# Autodesk Inventor assembly: Trunk
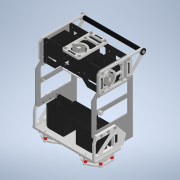
[picture p0: Inventor's stored thumbnail of the model, 180x180]
Saved by Autodesk Inventor 2020.4 (Build 244396000, 396)
## iProperties
Created: 2022-01-05
Part Number: Trunk
Document SubType Name: Assembly
Designer: Masato Kubotera
Author: Masato Kubotera
## Documents named in this file (25)
- C:\Users\Masato\Documents\Inventor\CIT Brains_Inventor\OpenPlatform_ver3_0 - ve4_1 branch\UpperBody\Trunk\Trunk.iam
- C:\Users\Masato\Documents\Inventor\CIT Brains_Inventor\OpenPlatform_ver3_0 - ve4_1 branch\Ready_Made\KONDO\B3M-SC-1040-A.ipt
- C:\Users\Masato\Documents\Inventor\CIT Brains_Inventor\OpenPlatform_ver3_0 - ve4_1 branch\Ready_Made\KONDO\B3M-SC-1170-A.ipt
- C:\Users\Masato\Documents\Inventor\CIT Brains_Inventor\OpenPlatform_ver3_0 - ve4_1 branch\UpperBody\Trunk\Trunk_chest_frame.ipt
- C:\Users\Masato\Documents\Inventor\CIT Brains_Inventor\OpenPlatform_ver3_0 - ve4_1 branch\Ready_Made\InsertNut\IRU-304SW.ipt
- C:\Users\Masato\Documents\Inventor\CIT Brains_Inventor\OpenPlatform_ver3_0 - ve4_1 branch\UpperBody\Trunk\Trunk_neck_Upper_frame.ipt
- C:\Users\Masato\Documents\Inventor\CIT Brains_Inventor\OpenPlatform_ver3_0 - ve4_1 branch\Ready_Made\Screw\M2_6-15.ipt
- C:\Users\Masato\Documents\Inventor\CIT Brains_Inventor\OpenPlatform_ver3_0 - ve4_1 branch\Ready_Made\Screw\M3-6.ipt
- C:\Users\Masato\Documents\Inventor\CIT Brains_Inventor\OpenPlatform_ver3_0 - ve4_1 branch\Ready_Made\Screw\M3-8.ipt
- C:\Users\Masato\Documents\Inventor\CIT Brains_Inventor\OpenPlatform_ver3_0 - ve4_1 branch\UpperBody\Trunk\Trunk_shoulder_frame_.ipt
- C:\Users\Masato\Documents\Inventor\CIT Brains_Inventor\OpenPlatform_ver3_0 - ve4_1 branch\UpperBody\Trunk\Trunk_upper_side_frame.ipt
- C:\Users\Masato\Documents\Inventor\CIT Brains_Inventor\OpenPlatform_ver3_0 - ve4_1 branch\Ready_Made\Screw\M3-10.ipt
- C:\Users\Masato\Documents\Inventor\CIT Brains_Inventor\OpenPlatform_ver3_0 - ve4_1 branch\Ready_Made\ABLSBF7-133-M3-N3.ipt
- C:\Users\Masato\Documents\Inventor\CIT Brains_Inventor\OpenPlatform_ver3_0 - ve4_1 branch\UpperBody\Trunk\Trunk_shoulder_frame_MIR.ipt
- C:\Users\Masato\Documents\Inventor\CIT Brains_Inventor\OpenPlatform_ver3_0 - ve4_1 branch\Ready_Made\UUW-0312-10BH.ipt
- C:\Users\Masato\Documents\Inventor\CIT Brains_Inventor\OpenPlatform_ver3_0 - ve4_1 branch\UpperBody\Trunk\Trunk_lower_side_frame.ipt
- C:\Users\Masato\Documents\Inventor\CIT Brains_Inventor\OpenPlatform_ver3_0 - ve4_1 branch\UpperBody\Trunk\Trunk_waisit_frame_.ipt
- C:\Users\Masato\Documents\Inventor\CIT Brains_Inventor\OpenPlatform_ver3_0 - ve4_1 branch\UpperBody\Trunk\CrossRollerBearing\BearingUnit.iam
- C:\Users\Masato\Documents\Inventor\CIT Brains_Inventor\OpenPlatform_ver3_0 - ve4_1 branch\Ready_Made\KONDO\ClampHorn.ipt
- C:\Users\Masato\Documents\Inventor\CIT Brains_Inventor\OpenPlatform_ver3_0 - ve4_1 branch\UpperBody\Trunk\Trunk_neck_lower_frame.ipt
- C:\Users\Masato\Documents\Inventor\CIT Brains_Inventor\OpenPlatform_ver3_0 - ve4_1 branch\UpperBody\Trunk\Trunk_waisit_diagonal.ipt
- C:\Users\Masato\Documents\Inventor\CIT Brains_Inventor\OpenPlatform_ver3_0 - ve4_1 branch\UpperBody\Trunk\Trunk_back_waisit_frame_.ipt
- C:\Users\Masato\Documents\Inventor\CIT Brains_Inventor\OpenPlatform_ver3_0 - ve4_1 branch\Ready_Made\KONDO\ClampHorn_Screw.ipt
- C:\Users\Masato\Documents\Inventor\CIT Brains_Inventor\OpenPlatform_ver3_0 - ve4_1 branch\Ready_Made\Screw\SPNFL-BRN-M3-6.ipt
- ClampHorn.ipt
## Components (91 placed, 23 different names)
1. B3M-SC-1040-A:1 — 挿入:13, 挿入:14, 挿入:15, 挿入:16, 挿入:95, 角度:2, 挿入:116
2. ClampHorn:1 — 挿入:95, 角度:2
3. B3M-SC-1040-A:2 — 挿入:41, 挿入:42, 挿入:43, 挿入:44, 挿入:96, 角度:3, 挿入:117
4. ClampHorn:2 — 挿入:96, 角度:3
5. B3M-SC-1040-A:3 — 挿入:61, 挿入:62, 挿入:63, 挿入:64, 挿入:97, 角度:4, 挿入:118
6. ClampHorn:3 — 挿入:97, 角度:4
7. B3M-SC-1170-A:1 — 挿入:87, 挿入:88
8. B3M-SC-1170-A:2 — 挿入:89, 挿入:90
9. Trunk_chest_frame:1 — 挿入:2, 挿入:3, 挿入:4, 挿入:6, 挿入:104, 挿入:105, 挿入:131
10. Trunk_chest_frame:2 — 挿入:7, 挿入:9, 挿入:10, 挿入:11, 挿入:12, 挿入:8, 挿入:102, 挿入:103
11. Trunk_neck_Upper_frame:1 — 挿入:13, 挿入:14, 挿入:15, 挿入:16, 挿入:18, 挿入:20, 挿入:21, 挿入:22, 挿入:23, 挿入:24, 挿入:25, 挿入:26, 挿入:27, 挿入:28
12. Trunk_upper_side_frame:1 — 挿入:29, 挿入:30, 挿入:31, 挿入:32, 挿入:33, 挿入:34, 挿入:35, 挿入:36, 挿入:5, 挿入:98, 挿入:99, 挿入:115, 挿入:119
13. Trunk_neck_lower_frame:1 — 挿入:106, 挿入:107, 挿入:108, 挿入:109, 挿入:110, 挿入:111, 挿入:112, 挿入:113
14. Trunk_shoulder_frame_:1 — 挿入:33, 挿入:34, 挿入:35, 挿入:36, 挿入:37, 挿入:39, 挿入:38, 挿入:40, 挿入:41, 挿入:42, 挿入:43, 挿入:44, 挿入:47, 挿入:48, 挿入:49, 挿入:50, 角度:1, 挿入:51
15. ABLSBF7-133-M3-N3:1 — 角度:1, 挿入:51, 挿入:60, 挿入:73, 挿入:74
16. Trunk_upper_side_frame:2 — 挿入:52, 挿入:53, 挿入:54, 挿入:55, 挿入:56, 挿入:57, 挿入:58, 挿入:59, 挿入:100, 挿入:101, 挿入:114, 挿入:120
17. Trunk_shoulder_frame_MIR:1 — 挿入:56, 挿入:57, 挿入:58, 挿入:59, 挿入:60, 挿入:61, 挿入:62, 挿入:63, 挿入:64, 挿入:65, 挿入:66, 挿入:67, 挿入:68, 挿入:69, 挿入:70, 挿入:71, 挿入:72
18. UUW-0312-10BH:1 — 挿入:73, 挿入:75
19. UUW-0312-10BH:2 — 挿入:74, 挿入:76
20. Trunk_waisit_diagonal:1 — 挿入:114
21. Trunk_back_waisit_frame_:1 — 挿入:115
22. Trunk_lower_side_frame:1 — メイト:1, フラッシュ:5, フラッシュ:6, フラッシュ:7, 挿入:98, 挿入:99, 挿入:125, 挿入:126, 挿入:127
23. Trunk_lower_side_frame:2 — メイト:2, フラッシュ:6, フラッシュ:8, 挿入:100, 挿入:101, 挿入:128, 挿入:129, 挿入:130
24. Trunk_waisit_frame_:1 — フラッシュ:2, フラッシュ:3, フラッシュ:4, 挿入:83, 挿入:84, 挿入:85, 挿入:86, 挿入:87, 挿入:88, 挿入:89, 挿入:90, 挿入:91, 挿入:92, 挿入:93, 挿入:94, メイト:1, メイト:2, フラッシュ:5, フラッシュ:7, フラッシュ:8, 挿入:121, 挿入:122, 挿入:123, 挿入:124
25. BearingUnit:1 [sub-assembly] — 挿入:83, 挿入:84
26. BearingUnit:2 [sub-assembly] — 挿入:85, 挿入:86
27. M3-10:7 — 挿入:125
28. M3-10:8 — 挿入:126
29. M3-10:9 — 挿入:127
30. M3-10:10 — 挿入:128
31. M3-10:11 — 挿入:129
32. M3-10:12 — 挿入:130
33. M3-10:13 — 挿入:121
34. M3-10:14 — 挿入:122
35. M3-10:15 — 挿入:123
36. M3-10:16 — 挿入:124
37. SPNFL-BRN-M3-6:1 — 挿入:119
38. SPNFL-BRN-M3-6:2 — 挿入:120
39. M3-8:2 — 挿入:28
40. M3-8:1 — 挿入:27
41. M3-6:2 — 挿入:26
42. M3-6:1 — 挿入:25
43. M2_6-15:4 — 挿入:24
44. M2_6-15:3 — 挿入:23
45. M2_6-15:2 — 挿入:22
46. M2_6-15:1 — 挿入:21
47. M2_6-15:8 — 挿入:50
48. M2_6-15:7 — 挿入:49
49. M2_6-15:6 — 挿入:48
50. M2_6-15:5 — 挿入:47
51. M3-8:4 — 挿入:38
52. M3-8:3 — 挿入:37
53. M3-10:4 — 挿入:40
54. M3-10:3 — 挿入:39
55. M2_6-15:12 — 挿入:72
56. M2_6-15:11 — 挿入:71
57. M2_6-15:10 — 挿入:70
58. M2_6-15:9 — 挿入:69
59. M3-10:6 — 挿入:68
60. M3-10:5 — 挿入:67
61. M3-8:6 — 挿入:66
62. M3-8:5 — 挿入:65
63. M3-6:4 — 挿入:76
64. M3-6:3 — 挿入:75
65. M2_6-15:16 — 挿入:94
66. M2_6-15:15 — 挿入:93
67. M2_6-15:14 — 挿入:92
68. M2_6-15:13 — 挿入:91
69. M3-6:8 — 挿入:113
70. M3-6:7 — 挿入:112
71. M3-6:6 — 挿入:111
72. M3-6:5 — 挿入:110
73. ClampHorn_Screw:1 — 挿入:116
74. ClampHorn_Screw:2 — 挿入:117
75. ClampHorn_Screw:3 — 挿入:118
76. IRU-304SW:12 — 挿入:12, 挿入:53
77. IRU-304SW:11 — 挿入:11, 挿入:52
78. IRU-304SW:10 — 挿入:10, 挿入:30
79. IRU-304SW:9 — 挿入:9, 挿入:29
80. IRU-304SW:8 — 挿入:8
81. IRU-304SW:7 — 挿入:7, 挿入:18
82. IRU-304SW:6 — 挿入:6, 挿入:32
83. IRU-304SW:5 — 挿入:5, 挿入:31
84. IRU-304SW:4 — 挿入:4, 挿入:55
85. IRU-304SW:3 — 挿入:3, 挿入:54
86. IRU-304SW:2 — 挿入:2, 挿入:20
87. IRU-304SW:1 — 挿入:131
88. IRU-304SW:16 — 挿入:104, 挿入:109
89. IRU-304SW:15 — 挿入:105, 挿入:108
90. IRU-304SW:14 — 挿入:103, 挿入:106
91. IRU-304SW:13 — 挿入:102, 挿入:107
## Relationships (133: Insert 120, Flush 7, Angle 4, Mate 2)
- 挿入:2 [Insert]: Trunk_chest_frame:1 ↔ IRU-304SW:2
- 挿入:3 [Insert]: Trunk_chest_frame:1 ↔ IRU-304SW:3
- 挿入:4 [Insert]: Trunk_chest_frame:1 ↔ IRU-304SW:4
- 挿入:5 [Insert]: Trunk_upper_side_frame:1 ↔ IRU-304SW:5
- 挿入:6 [Insert]: Trunk_chest_frame:1 ↔ IRU-304SW:6
- 挿入:7 [Insert]: Trunk_chest_frame:2 ↔ IRU-304SW:7
- 挿入:8 [Insert]: Trunk_chest_frame:2 ↔ IRU-304SW:8
- 挿入:9 [Insert]: Trunk_chest_frame:2 ↔ IRU-304SW:9
- 挿入:10 [Insert]: Trunk_chest_frame:2 ↔ IRU-304SW:10
- 挿入:11 [Insert]: Trunk_chest_frame:2 ↔ IRU-304SW:11
- 挿入:12 [Insert]: Trunk_chest_frame:2 ↔ IRU-304SW:12
- 挿入:13 [Insert]: B3M-SC-1040-A:1 ↔ Trunk_neck_Upper_frame:1
- 挿入:14 [Insert]: B3M-SC-1040-A:1 ↔ Trunk_neck_Upper_frame:1
- 挿入:15 [Insert]: B3M-SC-1040-A:1 ↔ Trunk_neck_Upper_frame:1
- 挿入:16 [Insert]: B3M-SC-1040-A:1 ↔ Trunk_neck_Upper_frame:1
- 挿入:18 [Insert]: Trunk_neck_Upper_frame:1 ↔ IRU-304SW:7
- 挿入:20 [Insert]: Trunk_neck_Upper_frame:1 ↔ IRU-304SW:2
- 挿入:21 [Insert]: Trunk_neck_Upper_frame:1 ↔ M2_6-15:1
- 挿入:22 [Insert]: Trunk_neck_Upper_frame:1 ↔ M2_6-15:2
- 挿入:23 [Insert]: Trunk_neck_Upper_frame:1 ↔ M2_6-15:3
- 挿入:24 [Insert]: Trunk_neck_Upper_frame:1 ↔ M2_6-15:4
- 挿入:25 [Insert]: Trunk_neck_Upper_frame:1 ↔ M3-6:1
- 挿入:26 [Insert]: Trunk_neck_Upper_frame:1 ↔ M3-6:2
- 挿入:27 [Insert]: Trunk_neck_Upper_frame:1 ↔ M3-8:1
- 挿入:28 [Insert]: Trunk_neck_Upper_frame:1 ↔ M3-8:2
- 挿入:29 [Insert]: Trunk_upper_side_frame:1 ↔ IRU-304SW:9
- 挿入:30 [Insert]: Trunk_upper_side_frame:1 ↔ IRU-304SW:10
- 挿入:31 [Insert]: Trunk_upper_side_frame:1 ↔ IRU-304SW:5
- 挿入:32 [Insert]: Trunk_upper_side_frame:1 ↔ IRU-304SW:6
- 挿入:33 [Insert]: Trunk_upper_side_frame:1 ↔ Trunk_shoulder_frame_:1
- 挿入:34 [Insert]: Trunk_upper_side_frame:1 ↔ Trunk_shoulder_frame_:1
- 挿入:35 [Insert]: Trunk_upper_side_frame:1 ↔ Trunk_shoulder_frame_:1
- 挿入:36 [Insert]: Trunk_upper_side_frame:1 ↔ Trunk_shoulder_frame_:1
- 挿入:37 [Insert]: Trunk_shoulder_frame_:1 ↔ M3-8:3
- 挿入:39 [Insert]: Trunk_shoulder_frame_:1 ↔ M3-10:3
- 挿入:38 [Insert]: Trunk_shoulder_frame_:1 ↔ M3-8:4
- 挿入:40 [Insert]: Trunk_shoulder_frame_:1 ↔ M3-10:4
- 挿入:41 [Insert]: B3M-SC-1040-A:2 ↔ Trunk_shoulder_frame_:1
- 挿入:42 [Insert]: B3M-SC-1040-A:2 ↔ Trunk_shoulder_frame_:1
- 挿入:43 [Insert]: B3M-SC-1040-A:2 ↔ Trunk_shoulder_frame_:1
- 挿入:44 [Insert]: B3M-SC-1040-A:2 ↔ Trunk_shoulder_frame_:1
- 挿入:47 [Insert]: Trunk_shoulder_frame_:1 ↔ M2_6-15:5
- 挿入:48 [Insert]: Trunk_shoulder_frame_:1 ↔ M2_6-15:6
- 挿入:49 [Insert]: Trunk_shoulder_frame_:1 ↔ M2_6-15:7
- 挿入:50 [Insert]: Trunk_shoulder_frame_:1 ↔ M2_6-15:8
- 角度:1 [Angle] (0 deg): Trunk_shoulder_frame_:1 ↔ ABLSBF7-133-M3-N3:1
- 挿入:51 [Insert]: Trunk_shoulder_frame_:1 ↔ ABLSBF7-133-M3-N3:1
- 挿入:52 [Insert]: Trunk_upper_side_frame:2 ↔ IRU-304SW:11
- 挿入:53 [Insert]: Trunk_upper_side_frame:2 ↔ IRU-304SW:12
- 挿入:54 [Insert]: Trunk_upper_side_frame:2 ↔ IRU-304SW:3
- 挿入:55 [Insert]: Trunk_upper_side_frame:2 ↔ IRU-304SW:4
- 挿入:56 [Insert]: Trunk_upper_side_frame:2 ↔ Trunk_shoulder_frame_MIR:1
- 挿入:57 [Insert]: Trunk_upper_side_frame:2 ↔ Trunk_shoulder_frame_MIR:1
- 挿入:58 [Insert]: Trunk_upper_side_frame:2 ↔ Trunk_shoulder_frame_MIR:1
- 挿入:59 [Insert]: Trunk_upper_side_frame:2 ↔ Trunk_shoulder_frame_MIR:1
- 挿入:60 [Insert]: ABLSBF7-133-M3-N3:1 ↔ Trunk_shoulder_frame_MIR:1
- 挿入:61 [Insert]: B3M-SC-1040-A:3 ↔ Trunk_shoulder_frame_MIR:1
- 挿入:62 [Insert]: B3M-SC-1040-A:3 ↔ Trunk_shoulder_frame_MIR:1
- 挿入:63 [Insert]: B3M-SC-1040-A:3 ↔ Trunk_shoulder_frame_MIR:1
- 挿入:64 [Insert]: B3M-SC-1040-A:3 ↔ Trunk_shoulder_frame_MIR:1
- 挿入:65 [Insert]: Trunk_shoulder_frame_MIR:1 ↔ M3-8:5
- 挿入:66 [Insert]: Trunk_shoulder_frame_MIR:1 ↔ M3-8:6
- 挿入:67 [Insert]: Trunk_shoulder_frame_MIR:1 ↔ M3-10:5
- 挿入:68 [Insert]: Trunk_shoulder_frame_MIR:1 ↔ M3-10:6
- 挿入:69 [Insert]: Trunk_shoulder_frame_MIR:1 ↔ M2_6-15:9
- 挿入:70 [Insert]: Trunk_shoulder_frame_MIR:1 ↔ M2_6-15:10
- 挿入:71 [Insert]: Trunk_shoulder_frame_MIR:1 ↔ M2_6-15:11
- 挿入:72 [Insert]: Trunk_shoulder_frame_MIR:1 ↔ M2_6-15:12
- 挿入:73 [Insert]: ABLSBF7-133-M3-N3:1 ↔ UUW-0312-10BH:1
- 挿入:74 [Insert]: ABLSBF7-133-M3-N3:1 ↔ UUW-0312-10BH:2
- 挿入:75 [Insert]: UUW-0312-10BH:1 ↔ M3-6:3
- 挿入:76 [Insert]: UUW-0312-10BH:2 ↔ M3-6:4
- フラッシュ:2 [Flush]: Trunk_waisit_frame_:1
- フラッシュ:3 [Flush]: Trunk_waisit_frame_:1
- フラッシュ:4 [Flush]: Trunk_waisit_frame_:1
- 挿入:83 [Insert]: Trunk_waisit_frame_:1 ↔ BearingUnit:1
- 挿入:84 [Insert]: Trunk_waisit_frame_:1 ↔ BearingUnit:1
- 挿入:85 [Insert]: Trunk_waisit_frame_:1 ↔ BearingUnit:2
- 挿入:86 [Insert]: Trunk_waisit_frame_:1 ↔ BearingUnit:2
- 挿入:87 [Insert]: B3M-SC-1170-A:1 ↔ Trunk_waisit_frame_:1
- 挿入:88 [Insert]: B3M-SC-1170-A:1 ↔ Trunk_waisit_frame_:1
- 挿入:89 [Insert]: B3M-SC-1170-A:2 ↔ Trunk_waisit_frame_:1
- 挿入:90 [Insert]: B3M-SC-1170-A:2 ↔ Trunk_waisit_frame_:1
- 挿入:91 [Insert]: Trunk_waisit_frame_:1 ↔ M2_6-15:13
- 挿入:92 [Insert]: Trunk_waisit_frame_:1 ↔ M2_6-15:14
- 挿入:93 [Insert]: Trunk_waisit_frame_:1 ↔ M2_6-15:15
- 挿入:94 [Insert]: Trunk_waisit_frame_:1 ↔ M2_6-15:16
- 挿入:95 [Insert]: B3M-SC-1040-A:1 ↔ ClampHorn:1
- 挿入:96 [Insert]: B3M-SC-1040-A:2 ↔ ClampHorn:2
- 挿入:97 [Insert]: B3M-SC-1040-A:3 ↔ ClampHorn:3
- 角度:2 [Angle] (0 deg): B3M-SC-1040-A:1 ↔ ClampHorn:1
- 角度:3 [Angle] (0 deg): B3M-SC-1040-A:2 ↔ ClampHorn:2
- 角度:4 [Angle] (0 deg): B3M-SC-1040-A:3 ↔ ClampHorn:3
- メイト:1 [Mate]: Trunk_lower_side_frame:1 ↔ Trunk_waisit_frame_:1
- メイト:2 [Mate]: Trunk_lower_side_frame:2 ↔ Trunk_waisit_frame_:1
- フラッシュ:5 [Flush]: Trunk_lower_side_frame:1 ↔ Trunk_waisit_frame_:1
- フラッシュ:6 [Flush]: Trunk_lower_side_frame:1 ↔ Trunk_lower_side_frame:2
- フラッシュ:7 [Flush] (2.5 mm): Trunk_lower_side_frame:1 ↔ Trunk_waisit_frame_:1
- フラッシュ:8 [Flush] (-2.5 mm): Trunk_lower_side_frame:2 ↔ Trunk_waisit_frame_:1
- 挿入:98 [Insert]: Trunk_upper_side_frame:1 ↔ Trunk_lower_side_frame:1
- 挿入:99 [Insert]: Trunk_upper_side_frame:1 ↔ Trunk_lower_side_frame:1
- 挿入:100 [Insert]: Trunk_upper_side_frame:2 ↔ Trunk_lower_side_frame:2
- 挿入:101 [Insert]: Trunk_upper_side_frame:2 ↔ Trunk_lower_side_frame:2
- 挿入:102 [Insert]: Trunk_chest_frame:2 ↔ IRU-304SW:13
- 挿入:103 [Insert]: Trunk_chest_frame:2 ↔ IRU-304SW:14
- 挿入:104 [Insert]: Trunk_chest_frame:1 ↔ IRU-304SW:16
- 挿入:105 [Insert]: Trunk_chest_frame:1 ↔ IRU-304SW:15
- 挿入:106 [Insert]: Trunk_neck_lower_frame:1 ↔ IRU-304SW:14
- 挿入:107 [Insert]: Trunk_neck_lower_frame:1 ↔ IRU-304SW:13
- 挿入:108 [Insert]: Trunk_neck_lower_frame:1 ↔ IRU-304SW:15
- 挿入:109 [Insert]: Trunk_neck_lower_frame:1 ↔ IRU-304SW:16
- 挿入:110 [Insert]: Trunk_neck_lower_frame:1 ↔ M3-6:5
- 挿入:111 [Insert]: Trunk_neck_lower_frame:1 ↔ M3-6:6
- 挿入:112 [Insert]: Trunk_neck_lower_frame:1 ↔ M3-6:7
- 挿入:113 [Insert]: Trunk_neck_lower_frame:1 ↔ M3-6:8
- 挿入:114 [Insert]: Trunk_upper_side_frame:2 ↔ Trunk_waisit_diagonal:1
- 挿入:115 [Insert]: Trunk_upper_side_frame:1 ↔ Trunk_back_waisit_frame_:1
- 挿入:116 [Insert]: B3M-SC-1040-A:1 ↔ ClampHorn_Screw:1
- 挿入:117 [Insert]: B3M-SC-1040-A:2 ↔ ClampHorn_Screw:2
- 挿入:118 [Insert]: B3M-SC-1040-A:3 ↔ ClampHorn_Screw:3
- 挿入:119 [Insert]: Trunk_upper_side_frame:1 ↔ SPNFL-BRN-M3-6:1
- 挿入:120 [Insert]: Trunk_upper_side_frame:2 ↔ SPNFL-BRN-M3-6:2
- 挿入:121 [Insert]: Trunk_waisit_frame_:1 ↔ M3-10:13
- 挿入:122 [Insert]: Trunk_waisit_frame_:1 ↔ M3-10:14
- 挿入:123 [Insert]: Trunk_waisit_frame_:1 ↔ M3-10:15
- 挿入:124 [Insert]: Trunk_waisit_frame_:1 ↔ M3-10:16
- 挿入:125 [Insert]: Trunk_lower_side_frame:1 ↔ M3-10:7
- 挿入:126 [Insert]: Trunk_lower_side_frame:1 ↔ M3-10:8
- 挿入:127 [Insert]: Trunk_lower_side_frame:1 ↔ M3-10:9
- 挿入:128 [Insert]: Trunk_lower_side_frame:2 ↔ M3-10:10
- 挿入:129 [Insert]: Trunk_lower_side_frame:2 ↔ M3-10:11
- 挿入:130 [Insert]: Trunk_lower_side_frame:2 ↔ M3-10:12
- 挿入:131 [Insert]: Trunk_chest_frame:1 ↔ IRU-304SW:1
